# Autodesk Inventor assembly: caster wheel v5
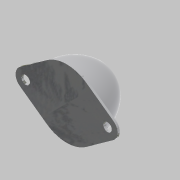
[picture p0: Inventor's stored thumbnail of the model, 180x180]
Saved by Autodesk Inventor 2019.3 (Build 233278000, 278)
## iProperties
Created: 2019-03-27
Part Number: caster wheel v5
Document SubType Name: Assembly
Designer: Varga Daniel
Author: Varga Daniel
## Documents named in this file (3)
- C:\!_Dani\!_cloud\OneDrive\!_munka\Revolution\RevvyDemoKit\Structural parts\Demo parts\Caster wheel\Inventor imported\caster wheel v5.iam
- C:\!_Dani\!_cloud\OneDrive\!_munka\Revolution\RevvyDemoKit\Structural parts\Demo parts\Caster wheel\Inventor imported\caster_wheel_v5_ball.ipt
- C:\!_Dani\!_cloud\OneDrive\!_munka\Revolution\RevvyDemoKit\Structural parts\Demo parts\Caster wheel\Inventor imported\caster_wheel_v5_base.ipt
## Components (2 placed, 2 different names)
1. caster_wheel_v5_ball:1 — Mate:1, Tangent:1
2. caster_wheel_v5_base:1 — Mate:1, Angle:1, Mate:2
## Relationships (4: Mate 2, Angle 1, Tangent 1)
- Mate:1: caster_wheel_v5_ball:1 ↔ caster_wheel_v5_base:1
- Angle:1 (0 deg): caster_wheel_v5_base:1
- Tangent:1: caster_wheel_v5_ball:1
- Mate:2 (-20 mm): caster_wheel_v5_base:1
